# Autodesk Inventor assembly: ASY PNS 1740 funnel
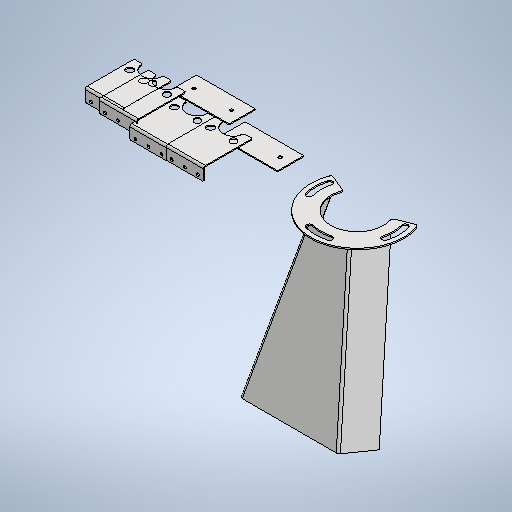
[picture p0: Inventor's stored thumbnail of the model, 512x512]
Saved by Autodesk Inventor 2025.3 (Build 293356030, 356C)
## iProperties
Created: 2025-09-12
Part Number: ASY PNS 1740 funnel
Document SubType Name: Assembly
Designer: admin
Author: admin
## Documents named in this file (5)
- C:\Users\admin\Yandex.Disk\home pc\Inventor\PNS2-Panaevsk\Filter D1200\ASY PNS 1740 funnel.iam
- C:\Users\admin\Yandex.Disk\home pc\Inventor\PNS2-Panaevsk\Filter D1200\PNS 1707 funnel flange .ipt
- C:\Users\admin\Yandex.Disk\home pc\Inventor\PNS2-Panaevsk\Filter D1200\PNS 1708 funnel body.ipt
- C:\Users\admin\Yandex.Disk\home pc\Inventor\PNS2-Panaevsk\PNS 2114 cyclone plate.ipt
- C:\Users\admin\Yandex.Disk\home pc\Inventor\Workshop\крючки уши кронштейны\nord 1.ipt
## Components (8 placed, 4 different names)
1. PNS 1707 funnel flange :1 — Mate:1, Mate:3
2. PNS 1708 funnel body:1 — Mate:1, Mate:2, Mate:3
3. PNS 2114 cyclone plate:1
4. PNS 2114 cyclone plate:2
5. Part1:1
6. Part1:2
7. Part1:3
8. Part1:4
## Relationships (3: Mate 3)
- Mate:1: PNS 1707 funnel flange :1 ↔ PNS 1708 funnel body:1
- Mate:2: PNS 1708 funnel body:1
- Mate:3: PNS 1707 funnel flange :1 ↔ PNS 1708 funnel body:1
